# Autodesk Inventor assembly: LaundryRobot_v01
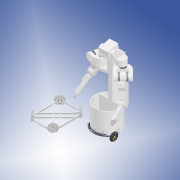
[picture p0: Inventor's stored thumbnail of the model, 180x180]
Saved by Autodesk Inventor 2017 SP1 (Build 210196100, 196)
## iProperties
Created: 2017-03-11
Part Number: LaundryRobot_v01
Document SubType Name: Assembly
Designer: zallen
Author: zallen
## Documents named in this file (5)
- C:\Users\Zach\Documents\GitHub\cr-laundry-robot\LaundryRobot_v01.iam
- C:\Users\Zach\Documents\GitHub\cr-laundry-robot\src\Base\Base.iam
- C:\Users\Zach\Documents\GitHub\cr-laundry-robot\src\Body\Body.iam
- C:\Users\Zach\Documents\GitHub\cr-laundry-robot\src\Head\Head.iam
- C:\Users\Zach\Documents\GitHub\cr-laundry-robot\src\Base 2\Base2.iam
## Components (4 placed, 4 different names)
1. Base:1 [sub-assembly] — Mate:1, Mate:2, Mate:4, Mate:5, Mate:6
2. Body:1 [sub-assembly] — Mate:1, Mate:2, Mate:7, Mate:8, Mate:9
3. Head:1 [sub-assembly] — Mate:7, Mate:8, Mate:9
4. Base2:1 [sub-assembly] — Mate:10, Mate:11
## Relationships (10: Mate 10)
- Mate:1: Base:1 ↔ Body:1
- Mate:2: Base:1 ↔ Body:1
- Mate:4: Base:1
- Mate:5: Base:1
- Mate:6: Base:1
- Mate:7: Body:1 ↔ Head:1
- Mate:8: Body:1 ↔ Head:1
- Mate:9: Body:1 ↔ Head:1
- Mate:10: Base2:1
- Mate:11: Base2:1
